# Autodesk Inventor assembly: Fence generator - assembly level one-02
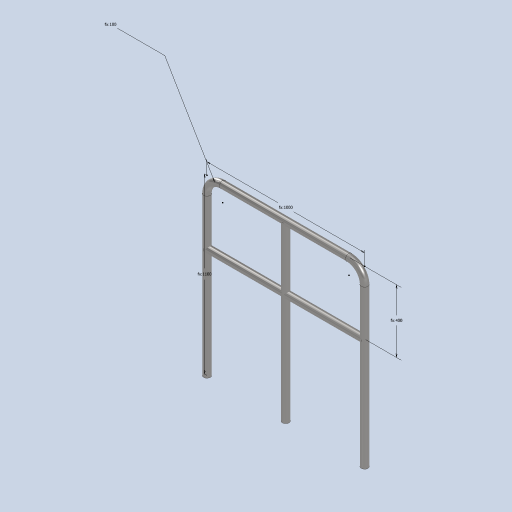
[picture p0: Inventor's stored thumbnail of the model, 512x512]
Saved by Autodesk Inventor 2024.3 (Build 283343000, 343)
## iProperties
RuleStatus: InUse
AfterDocNew0: Fence generator - sketch-01 Rule
Created: 2024-08-12
Part Number: Fence generator - assembly level one-02
Document SubType Name: Assembly
Designer: MPA
fenceW: 1000,000 mm
fenceL: 1100,000 mm
filetSize: 100,000 mm
middleDist: 400,000 mm
_SolveAssemblyDoc: Frame Generator Solve Assembly
_Version: 15.0.0
Author: MPA
## Documents named in this file (3)
- C:\Users\Public\Documents\Autodesk\Inventor 2024\Templates\en-US\Metric\Balustrady - test\Fence generator - assembly level one.iam
- C:\MPA - shortPath\Balustrady - test\Fence generator - sketch-01.ipt
- C:\Users\Public\Documents\Autodesk\Inventor 2024\Templates\en-US\Metric\Balustrady - test\Fence generator - assembly level one\Frame\Frame 1723491092086.iam
## Components (2 placed, 2 different names)
1. Fence generator - sketch-01:1 — Flush:1, Flush:2, Flush:3
2. Frame 1723491092086:1 [sub-assembly]
## Relationships (3: Flush 3)
- Flush:1: Fence generator - sketch-01:1
- Flush:2: Fence generator - sketch-01:1
- Flush:3: Fence generator - sketch-01:1
